# Autodesk Inventor assembly: Surge Arrester
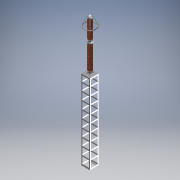
[picture p0: Inventor's stored thumbnail of the model, 180x180]
Saved by Autodesk Inventor 2016 (Build 200138000, 138)
## iProperties
Created: 2017-01-19
Part Number: Surge Arrester
Document SubType Name: Assembly
Designer: admin
Author: admin
## Documents named in this file (3)
- C:\Users\admin\Documents\ITER INV\Patio 400kV\Surge Arrester PPEN\Surge Arrester.iam
- C:\Users\admin\Documents\ITER INV\Patio 400kV\Surge Arrester PPEN\Celosia.ipt
- C:\Users\admin\Documents\ITER INV\Patio 400kV\Surge Arrester PPEN\Surge Arrester Esc.ipt
## Components (2 placed, 2 different names)
1. Celosia:1 — Mate:1, Flush:1, Mate:3, Angle:1, Mate:4
2. Surge Arrester Esc:1 — Flush:1, Mate:3, Angle:1, Mate:4
## Relationships (5: Mate 3, Flush 1, Angle 1)
- Mate:1: Celosia:1
- Flush:1: Celosia:1 ↔ Surge Arrester Esc:1
- Mate:3: Celosia:1 ↔ Surge Arrester Esc:1
- Angle:1 (0 deg): Celosia:1 ↔ Surge Arrester Esc:1
- Mate:4: Celosia:1 ↔ Surge Arrester Esc:1
